# Autodesk Inventor assembly: 608ZZ
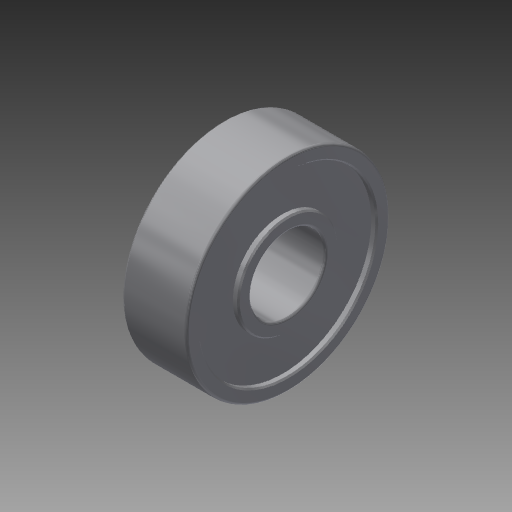
[picture p0: Inventor's stored thumbnail of the model, 512x512]
Saved by Autodesk Inventor 2018 (Build 220112000, 112)
## iProperties
Created: 2018-01-21
Part Number: 608ZZ
Description: STEP AP214
Document SubType Name: Assembly
Designer: Rus
Sending System: PARTsolutions
Preprocessor: PSStep 15.0.47
Title: //expscmdclustefs.cadenas.external/client_exchange/iodir/jobs/output/wkb78934751_no0/STEP/608ZZ_2_14b.stp
Revision Number: NONE
## Documents named in this file (6)
- E:\Libraries\3D Objects\Geneva drive\Mechanical\Attempt 2v2\608ZZ.iam
- E:\Libraries\3D Objects\Geneva drive\Mechanical\Attempt 2v2\_608ZZ_ir.ipt
- E:\Libraries\3D Objects\Geneva drive\Mechanical\Attempt 2v2\_608ZZ_cage.ipt
- E:\Libraries\3D Objects\Geneva drive\Mechanical\Attempt 2v2\_608ZZ_ball.ipt
- E:\Libraries\3D Objects\Geneva drive\Mechanical\Attempt 2v2\_608ZZ_or.ipt
- E:\Libraries\3D Objects\Geneva drive\Mechanical\Attempt 2v2\_608ZZ_shield.ipt
## Components (12 placed, 12 different names)
1. NAUO1 — Rotational:1, Insert:4
2. NAUO2 — Ball:1, Ball:2, Ball:3, Ball:4, Ball:5, Ball:6, Ball:7, Rotational:1
3. NAUO3 — Ball:6
4. NAUO4 — Ball:7
5. NAUO5 — Ball:3
6. NAUO6 — Ball:2
7. NAUO7 — Ball:1
8. NAUO8 — Ball:4
9. NAUO9 — Ball:5
10. NAUO10 — Insert:2, Insert:3, Insert:4
11. NAUO11 — Insert:3
12. NAUO12 — Insert:2
## Relationships (11: BallJoint 7, Insert 3, RevoluteJoint 1)
- Ball:1: NAUO2 ↔ NAUO7
- Ball:2: NAUO2 ↔ NAUO6
- Ball:3: NAUO2 ↔ NAUO5
- Ball:4: NAUO2 ↔ NAUO8
- Ball:5: NAUO2 ↔ NAUO9
- Ball:6: NAUO2 ↔ NAUO3
- Ball:7: NAUO2 ↔ NAUO4
- Rotational:1 [RevoluteJoint]: NAUO1 ↔ NAUO2
- Insert:2: NAUO10 ↔ NAUO12
- Insert:3: NAUO10 ↔ NAUO11
- Insert:4: NAUO1 ↔ NAUO10
